# Autodesk Inventor assembly: Drivebase AM14U4 Square 28inx28in v411
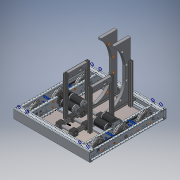
[picture p0: Inventor's stored thumbnail of the model, 180x180]
Saved by Autodesk Inventor 2018 (Build 220112000, 112)
## iProperties
Created: 2020-01-28
Part Number: Drivebase AM14U4 Square 28inx28in v411
Document SubType Name: Assembly
Designer: Weeb No1
Sending System: Autodesk Translation Framework v8.12.0.6
Preprocessor: ST-DEVELOPER v18
Title: /Users/GabG/Documents/GitHub/2020CAD/New Gabriel Shooter/Drivebase AM14U4 Square 28inx28in v41.step
## Documents named in this file (15)
- C:\Users\Weeb No1\Documents\GitHub\2020CAD\Gabriel Inventor Files (Shooter, Drivebase)\Drivebase Assembly\Main Assembly\Drivebase AM14U4 Square 28inx28in v411.iam
- C:\Users\Weeb No1\Documents\GitHub\2020CAD\Gabriel Inventor Files (Shooter, Drivebase)\Drivebase Assembly\Part Files\AM14U4 Square Half.iam
- C:\Users\Weeb No1\Documents\GitHub\2020CAD\Gabriel Inventor Files (Shooter, Drivebase)\Drivebase Assembly\Part Files\AM14U4 Square Half_1.iam
- C:\Users\Weeb No1\Documents\GitHub\2020CAD\Gabriel Inventor Files (Shooter, Drivebase)\Drivebase Assembly\Part Files\Placeholder Belly Pan.ipt
- C:\Users\Weeb No1\Documents\GitHub\2020CAD\Gabriel Inventor Files (Shooter, Drivebase)\Drivebase Assembly\Part Files\10-24 Washer.ipt
- C:\Users\Weeb No1\Documents\GitHub\2020CAD\Gabriel Inventor Files (Shooter, Drivebase)\Drivebase Assembly\Part Files\Bumper Assembly.iam
- C:\Users\Weeb No1\Documents\GitHub\2020CAD\Gabriel Inventor Files (Shooter, Drivebase)\Drivebase Assembly\Part Files\Bumper Assembly_1.iam
- C:\Users\Weeb No1\Documents\GitHub\2020CAD\Gabriel Inventor Files (Shooter, Drivebase)\Drivebase Assembly\Part Files\95335A503_METRIC QUICK-RELEASE PIN.ipt
- C:\Users\Weeb No1\Documents\GitHub\2020CAD\Gabriel Inventor Files (Shooter, Drivebase)\Drivebase Assembly\Part Files\8020 1010 x 26 v2.ipt
- C:\Users\Weeb No1\Documents\GitHub\2020CAD\Gabriel Inventor Files (Shooter, Drivebase)\Drivebase Assembly\Part Files\Component52.ipt
- C:\Users\Weeb No1\Documents\GitHub\2020CAD\Gabriel Inventor Files (Shooter, Drivebase)\Drivebase Assembly\Part Files\VersaBlock_Mini_Kit_217-5852.iam
- C:\Users\Weeb No1\Documents\GitHub\2020CAD\Gabriel Inventor Files (Shooter, Drivebase)\Drivebase Assembly\Part Files\8020 1010 x 6.ipt
- C:\Users\Weeb No1\Documents\GitHub\2020CAD\Gabriel Inventor Files (Shooter, Drivebase)\Shooter Curve Assembly\Main Assembly File\Shooter Curve Assembly.iam
- C:\Users\Weeb No1\Documents\GitHub\2020CAD\Tyler's Ball Storage\Other parts\am-0028 00.375'' id Flanged, Shielded Ball Bearing (FR6ZZ).ipt
- C:\Users\Weeb No1\Documents\GitHub\2020CAD\Tyler's Ball Storage\Polycarb half main conv.iam
## Components (39 placed, 14 different names)
1. AM14U4 Square Half:1 [sub-assembly] — Mate:69, Mate:70, Mate:71, Mate:75, Mate:76, Mate:77, Mate:82, Mate:83, Mate:84, Mate:85, Mate:91, Mate:92, Mate:96, Mate:97, Symmetry:1, Mate:198, Mate:199, Flush:75, Mate:209, Mate:214, Mate:215
2. AM14U4 Square Half_1:1 [sub-assembly] — Mate:66, Mate:67, Mate:68, Mate:72, Mate:73, Mate:74, Mate:78, Mate:79, Mate:80, Mate:81, Mate:93, Mate:94, Mate:95, Mate:98, Symmetry:1, Mate:203, Flush:77, Mate:206, Mate:208
3. Placeholder Belly Pan:1 — Mate:91, Mate:92, Mate:93, Mate:94, Mate:95, Mate:96, Mate:97, Mate:98, Mate:99, Mate:100, Mate:101, Mate:102, Mate:103, Mate:104, Mate:105, Mate:106, Mate:216, Mate:217
4. 10-24 Washer:1 — Mate:101
5. 10-24 Washer:2 — Mate:102
6. 10-24 Washer:3 — Mate:100
7. 10-24 Washer:4 — Mate:99
8. 10-24 Washer:5 — Mate:106
9. 10-24 Washer:6 — Mate:105
10. 10-24 Washer:7 — Mate:104
11. 10-24 Washer:8 — Mate:103
12. Bumper Assembly:1 [sub-assembly] — Mate:72, Mate:73, Mate:74, Mate:75, Mate:76, Mate:77
13. Bumper Assembly_1:1 [sub-assembly] — Mate:66, Mate:67, Mate:68, Mate:69, Mate:70, Mate:71
14. 95335A503_METRIC QUICK-RELEASE PIN:1 — Mate:82
15. 95335A503_METRIC QUICK-RELEASE PIN:2 — Mate:83
16. 95335A503_METRIC QUICK-RELEASE PIN:3 — Mate:85
17. 95335A503_METRIC QUICK-RELEASE PIN:4 — Mate:84
18. 95335A503_METRIC QUICK-RELEASE PIN:5 — Mate:78
19. 95335A503_METRIC QUICK-RELEASE PIN:6 — Mate:79
20. 95335A503_METRIC QUICK-RELEASE PIN:7 — Mate:80
21. 95335A503_METRIC QUICK-RELEASE PIN:8 — Mate:81
22. 8020 1010 x 26 v2:1 — Mate:198, Flush:76, Mate:202, Flush:80, Mate:210, Mate:211, Mate:212, Flush:81, Mate:234, Mate:235, Mate:236, Mate:237, Mate:238, Mate:239
23. 8020 1010 x 26 v2:2 — Mate:206, Mate:207, Flush:78, Flush:79, Mate:213, Flush:82
24. Component52:1
25. VersaBlock_Mini_Kit_217-5852:1 [sub-assembly] — Mate:210, Mate:211
26. 8020 1010 x 6:1 — Mate:203, Flush:77, Mate:207, Flush:78, Flush:80
27. 8020 1010 x 6:2 — Mate:199, Flush:75, Flush:76, Mate:202, Mate:208, Mate:209, Flush:79
28. Shooter Curve Assembly:1 [sub-assembly] — Mate:212, Mate:213, Mate:214, Mate:215, Flush:81, Flush:82, Mate:216, Mate:217, Mate:218, Mate:219, Mate:220, Mate:221, Mate:222, Mate:223, Mate:224, Mate:225, Mate:226, Mate:227, Mate:228, Mate:229, Mate:230, Mate:231, Mate:232, Mate:233
29. am-0028 00.375'' id Flanged, Shielded Ball Bearing (FR6ZZ):1 — Mate:222, Mate:223
30. am-0028 00.375'' id Flanged, Shielded Ball Bearing (FR6ZZ):2 — Mate:220, Mate:221
31. am-0028 00.375'' id Flanged, Shielded Ball Bearing (FR6ZZ):3 — Mate:218, Mate:219
32. am-0028 00.375'' id Flanged, Shielded Ball Bearing (FR6ZZ):4 — Mate:224, Mate:225
33. am-0028 00.375'' id Flanged, Shielded Ball Bearing (FR6ZZ):5 — Mate:226, Mate:227
34. am-0028 00.375'' id Flanged, Shielded Ball Bearing (FR6ZZ):6 — Mate:228, Mate:229
35. am-0028 00.375'' id Flanged, Shielded Ball Bearing (FR6ZZ):7 — Mate:232, Mate:233
36. am-0028 00.375'' id Flanged, Shielded Ball Bearing (FR6ZZ):8 — Mate:230, Mate:231
37. Polycarb half main conv:1 [sub-assembly] — Mate:234, Mate:235
38. Polycarb half main conv:2 [sub-assembly] — Mate:236, Mate:237
39. Polycarb half main conv:3 [sub-assembly] — Mate:238, Mate:239
## Relationships (83: Mate 74, Flush 8, Symmetry 1)
- Mate:66: AM14U4 Square Half_1:1 ↔ Bumper Assembly_1:1
- Mate:67: AM14U4 Square Half_1:1 ↔ Bumper Assembly_1:1
- Mate:68: AM14U4 Square Half_1:1 ↔ Bumper Assembly_1:1
- Mate:69: AM14U4 Square Half:1 ↔ Bumper Assembly_1:1
- Mate:70: AM14U4 Square Half:1 ↔ Bumper Assembly_1:1
- Mate:71: AM14U4 Square Half:1 ↔ Bumper Assembly_1:1
- Mate:72: AM14U4 Square Half_1:1 ↔ Bumper Assembly:1
- Mate:73: AM14U4 Square Half_1:1 ↔ Bumper Assembly:1
- Mate:74: AM14U4 Square Half_1:1 ↔ Bumper Assembly:1
- Mate:75: AM14U4 Square Half:1 ↔ Bumper Assembly:1
- Mate:76: AM14U4 Square Half:1 ↔ Bumper Assembly:1
- Mate:77: AM14U4 Square Half:1 ↔ Bumper Assembly:1
- Mate:78: AM14U4 Square Half_1:1 ↔ 95335A503_METRIC QUICK-RELEASE PIN:5
- Mate:79: AM14U4 Square Half_1:1 ↔ 95335A503_METRIC QUICK-RELEASE PIN:6
- Mate:80: AM14U4 Square Half_1:1 ↔ 95335A503_METRIC QUICK-RELEASE PIN:7
- Mate:81: AM14U4 Square Half_1:1 ↔ 95335A503_METRIC QUICK-RELEASE PIN:8
- Mate:82: AM14U4 Square Half:1 ↔ 95335A503_METRIC QUICK-RELEASE PIN:1
- Mate:83: AM14U4 Square Half:1 ↔ 95335A503_METRIC QUICK-RELEASE PIN:2
- Mate:84: AM14U4 Square Half:1 ↔ 95335A503_METRIC QUICK-RELEASE PIN:4
- Mate:85: AM14U4 Square Half:1 ↔ 95335A503_METRIC QUICK-RELEASE PIN:3
- Mate:91: AM14U4 Square Half:1 ↔ Placeholder Belly Pan:1
- Mate:92: AM14U4 Square Half:1 ↔ Placeholder Belly Pan:1
- Mate:93: AM14U4 Square Half_1:1 ↔ Placeholder Belly Pan:1
- Mate:94: AM14U4 Square Half_1:1 ↔ Placeholder Belly Pan:1
- Mate:95: AM14U4 Square Half_1:1 ↔ Placeholder Belly Pan:1
- Mate:96: AM14U4 Square Half:1 ↔ Placeholder Belly Pan:1
- Mate:97: AM14U4 Square Half:1 ↔ Placeholder Belly Pan:1
- Mate:98: AM14U4 Square Half_1:1 ↔ Placeholder Belly Pan:1
- Mate:99: Placeholder Belly Pan:1 ↔ 10-24 Washer:4
- Mate:100: Placeholder Belly Pan:1 ↔ 10-24 Washer:3
- Mate:101: Placeholder Belly Pan:1 ↔ 10-24 Washer:1
- Mate:102: Placeholder Belly Pan:1 ↔ 10-24 Washer:2
- Mate:103: Placeholder Belly Pan:1 ↔ 10-24 Washer:8
- Mate:104: Placeholder Belly Pan:1 ↔ 10-24 Washer:7
- Mate:105: Placeholder Belly Pan:1 ↔ 10-24 Washer:6
- Mate:106: Placeholder Belly Pan:1 ↔ 10-24 Washer:5
- Symmetry:1: AM14U4 Square Half:1 ↔ AM14U4 Square Half_1:1
- Mate:198 (12.7 mm): AM14U4 Square Half:1 ↔ 8020 1010 x 26 v2:1
- Mate:199 (12.7 mm): AM14U4 Square Half:1 ↔ 8020 1010 x 6:2
- Flush:75 (5.588 mm): AM14U4 Square Half:1 ↔ 8020 1010 x 6:2
- Flush:76: 8020 1010 x 26 v2:1 ↔ 8020 1010 x 6:2
- Mate:202: 8020 1010 x 26 v2:1 ↔ 8020 1010 x 6:2
- Mate:203 (12.7 mm): AM14U4 Square Half_1:1 ↔ 8020 1010 x 6:1
- Flush:77 (5.588 mm): AM14U4 Square Half_1:1 ↔ 8020 1010 x 6:1
- Mate:206 (12.7 mm): AM14U4 Square Half_1:1 ↔ 8020 1010 x 26 v2:2
- Mate:207: 8020 1010 x 26 v2:2 ↔ 8020 1010 x 6:1
- Flush:78: 8020 1010 x 26 v2:2 ↔ 8020 1010 x 6:1
- Mate:208 (168.275 mm): AM14U4 Square Half_1:1 ↔ 8020 1010 x 6:2
- Mate:209 (168.275 mm): AM14U4 Square Half:1 ↔ 8020 1010 x 6:2
- Flush:79: 8020 1010 x 26 v2:2 ↔ 8020 1010 x 6:2
- Flush:80: 8020 1010 x 26 v2:1 ↔ 8020 1010 x 6:1
- Mate:210: 8020 1010 x 26 v2:1 ↔ VersaBlock_Mini_Kit_217-5852:1
- Mate:211: 8020 1010 x 26 v2:1 ↔ VersaBlock_Mini_Kit_217-5852:1
- Mate:212: 8020 1010 x 26 v2:1 ↔ Shooter Curve Assembly:1
- Mate:213: 8020 1010 x 26 v2:2 ↔ Shooter Curve Assembly:1
- Mate:214: AM14U4 Square Half:1 ↔ Shooter Curve Assembly:1
- Mate:215: AM14U4 Square Half:1 ↔ Shooter Curve Assembly:1
- Flush:81: 8020 1010 x 26 v2:1 ↔ Shooter Curve Assembly:1
- Flush:82: 8020 1010 x 26 v2:2 ↔ Shooter Curve Assembly:1
- Mate:216: Placeholder Belly Pan:1 ↔ Shooter Curve Assembly:1
- Mate:217: Placeholder Belly Pan:1 ↔ Shooter Curve Assembly:1
- Mate:218: Shooter Curve Assembly:1 ↔ am-0028 00.375'' id Flanged, Shielded Ball Bearing (FR6ZZ):3
- Mate:219: Shooter Curve Assembly:1 ↔ am-0028 00.375'' id Flanged, Shielded Ball Bearing (FR6ZZ):3
- Mate:220: Shooter Curve Assembly:1 ↔ am-0028 00.375'' id Flanged, Shielded Ball Bearing (FR6ZZ):2
- Mate:221: Shooter Curve Assembly:1 ↔ am-0028 00.375'' id Flanged, Shielded Ball Bearing (FR6ZZ):2
- Mate:222: Shooter Curve Assembly:1 ↔ am-0028 00.375'' id Flanged, Shielded Ball Bearing (FR6ZZ):1
- Mate:223: Shooter Curve Assembly:1 ↔ am-0028 00.375'' id Flanged, Shielded Ball Bearing (FR6ZZ):1
- Mate:224: Shooter Curve Assembly:1 ↔ am-0028 00.375'' id Flanged, Shielded Ball Bearing (FR6ZZ):4
- Mate:225: Shooter Curve Assembly:1 ↔ am-0028 00.375'' id Flanged, Shielded Ball Bearing (FR6ZZ):4
- Mate:226: Shooter Curve Assembly:1 ↔ am-0028 00.375'' id Flanged, Shielded Ball Bearing (FR6ZZ):5
- Mate:227: Shooter Curve Assembly:1 ↔ am-0028 00.375'' id Flanged, Shielded Ball Bearing (FR6ZZ):5
- Mate:228: Shooter Curve Assembly:1 ↔ am-0028 00.375'' id Flanged, Shielded Ball Bearing (FR6ZZ):6
- Mate:229: Shooter Curve Assembly:1 ↔ am-0028 00.375'' id Flanged, Shielded Ball Bearing (FR6ZZ):6
- Mate:230: Shooter Curve Assembly:1 ↔ am-0028 00.375'' id Flanged, Shielded Ball Bearing (FR6ZZ):8
- Mate:231: Shooter Curve Assembly:1 ↔ am-0028 00.375'' id Flanged, Shielded Ball Bearing (FR6ZZ):8
- Mate:232: Shooter Curve Assembly:1 ↔ am-0028 00.375'' id Flanged, Shielded Ball Bearing (FR6ZZ):7
- Mate:233: Shooter Curve Assembly:1 ↔ am-0028 00.375'' id Flanged, Shielded Ball Bearing (FR6ZZ):7
- Mate:234: 8020 1010 x 26 v2:1 ↔ Polycarb half main conv:1
- Mate:235: 8020 1010 x 26 v2:1 ↔ Polycarb half main conv:1
- Mate:236: 8020 1010 x 26 v2:1 ↔ Polycarb half main conv:2
- Mate:237: 8020 1010 x 26 v2:1 ↔ Polycarb half main conv:2
- Mate:238: 8020 1010 x 26 v2:1 ↔ Polycarb half main conv:3
- Mate:239: 8020 1010 x 26 v2:1 ↔ Polycarb half main conv:3
